# Autodesk Inventor assembly: vertical_mirrored
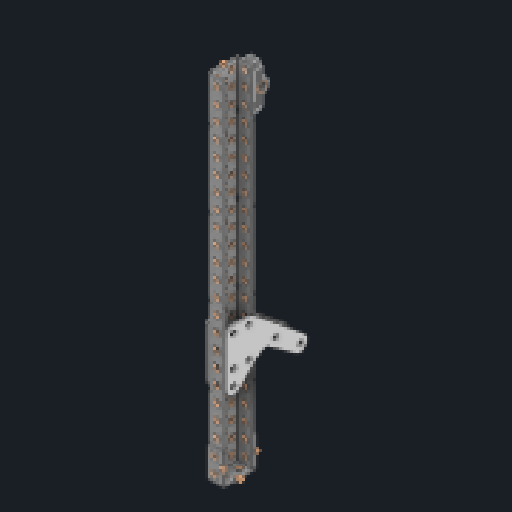
[picture p0: Inventor's stored thumbnail of the model, 512x512]
Saved by Autodesk Inventor 2025 (Build 290162000, 162)
## iProperties
Created: 2024-10-13
Part Number: vertical_mirrored
Document SubType Name: Assembly
Designer: Averey Ku
Author: Averey Ku
## Documents named in this file (5)
- D:\vex_robotics_high_stakes\hardware\cad\bots\high_stakes_v2\tower\structure\side_mirrored\vertical_mirrored.iam
- D:\vex_robotics_high_stakes\hardware\cad\bots\high_stakes_v2\tower\structure\side_mirrored\Alu C 2x2x2x1_mirrored.ipt
- D:\vex_robotics_high_stakes\hardware\cad\bots\high_stakes_v2\tower\structure\side_mirrored\Alu C 1x2x1x23_mirrored.ipt
- D:\vex_robotics_high_stakes\hardware\cad\bots\high_stakes_v2\tower\structure\side_mirrored\HS Pillow Bearing Block_mirrored.ipt
- D:\vex_robotics_high_stakes\hardware\cad\bots\high_stakes_v2\tower\structure\side_mirrored\triangle_brace_gusset_mirrored.ipt
## Components (5 placed, 4 different names)
1. Alu C 2x2x2x1_mirrored:1 — Mate:2, Insert:1, Mate:1
2. Alu C 1x2x1x23_mirrored:1 — Insert:1, Mate:1, Mate:5, Insert:4, Mate:7, Insert:6, Mate:8, Insert:7
3. HS Pillow Bearing Block_mirrored:1 — Mate:5, Insert:4
4. triangle_brace_gusset_mirrored:1 — Mate:7, Insert:6
5. triangle_brace_gusset_mirrored:2 — Mate:8, Insert:7
## Relationships (9: Mate 5, Insert 4)
- Mate:2: Alu C 2x2x2x1_mirrored:1
- Insert:1: Alu C 2x2x2x1_mirrored:1 ↔ Alu C 1x2x1x23_mirrored:1
- Mate:1: Alu C 2x2x2x1_mirrored:1 ↔ Alu C 1x2x1x23_mirrored:1
- Mate:5: Alu C 1x2x1x23_mirrored:1 ↔ HS Pillow Bearing Block_mirrored:1
- Insert:4: Alu C 1x2x1x23_mirrored:1 ↔ HS Pillow Bearing Block_mirrored:1
- Mate:7: Alu C 1x2x1x23_mirrored:1 ↔ triangle_brace_gusset_mirrored:1
- Insert:6: Alu C 1x2x1x23_mirrored:1 ↔ triangle_brace_gusset_mirrored:1
- Mate:8: Alu C 1x2x1x23_mirrored:1 ↔ triangle_brace_gusset_mirrored:2
- Insert:7 (12.7 mm): Alu C 1x2x1x23_mirrored:1 ↔ triangle_brace_gusset_mirrored:2
